# Autodesk Inventor assembly: FullCaseWithBaccable
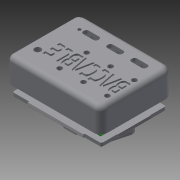
[picture p0: Inventor's stored thumbnail of the model, 180x180]
Saved by Autodesk Inventor 2014 SP2 (Build 180246200, 246)
## iProperties
Created: 2025-02-22
Part Number: FullCaseWithBaccable
Document SubType Name: Assembly
Designer: GauchoHP
Author: GauchoHP
## Documents named in this file (4)
- G:\Dati\Documenti_Emanuele\Linguaggi_di_Programmazione\ST MCU\baccable\canable\BACCAble-master\hardware\box\baccable_lastest_case_for_new_PCB\FullCaseWithBaccable.iam
- G:\Dati\Documenti_Emanuele\Linguaggi_di_Programmazione\ST MCU\baccable\canable\BACCAble-master\hardware\box\baccable_lastest_case_for_new_PCB\obdBase.ipt
- G:\Dati\Documenti_Emanuele\Linguaggi_di_Programmazione\ST MCU\baccable\canable\BACCAble-master\hardware\box\baccable_lastest_case_for_new_PCB\Imported Components\Baccable4\Baccable4.ipt
- G:\Dati\Documenti_Emanuele\Linguaggi_di_Programmazione\ST MCU\baccable\canable\BACCAble-master\hardware\box\baccable_lastest_case_for_new_PCB\cover.ipt
## Components (3 placed, 3 different names)
1. obdBase:1 — Mate:2, Mate:3, Flush:1, Flush:2, Mate:4
2. Baccable4:1 — Mate:2, Mate:3, Mate:4
3. cover:1 — Flush:1, Flush:2
## Relationships (5: Mate 3, Flush 2)
- Mate:2 (0.2 mm): obdBase:1 ↔ Baccable4:1
- Mate:3 (0.1 mm): obdBase:1 ↔ Baccable4:1
- Flush:1 (-1.8 mm): obdBase:1 ↔ cover:1
- Flush:2 (-2.8 mm): obdBase:1 ↔ cover:1
- Mate:4: obdBase:1 ↔ Baccable4:1
